# Autodesk Inventor assembly: Top_Separator Assy 3 Lanes
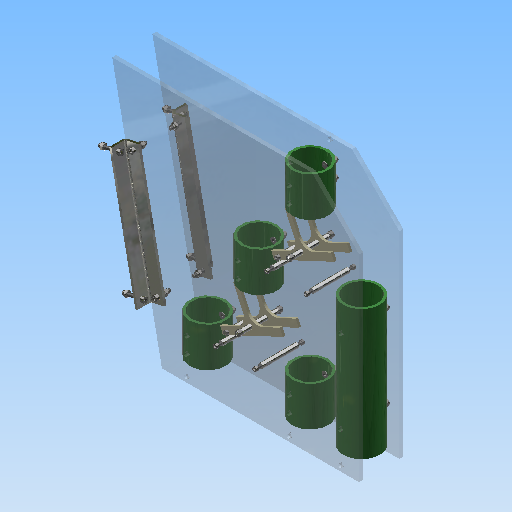
[picture p0: Inventor's stored thumbnail of the model, 512x512]
Saved by Autodesk Inventor 2018.1 (Build 221171000, 171)
## iProperties
Created: 2019-03-20
Part Number: Top_Separator Assy 3 Lanes
Document SubType Name: Assembly
Designer: James
Author: James
## Documents named in this file (16)
- C:\Users\admin\Desktop\Ball-Machine\Top Level\Top_Separator Assy 3 Lanes.iam
- C:\Users\admin\Desktop\Ball-Machine\Top Level\Top_Separator Pipe.ipt
- C:\Users\admin\Desktop\Ball-Machine\Top Level\Nyloc Nut - M4.ipt
- C:\Users\admin\Desktop\Ball-Machine\Top Level\Socket Csk Screw - (A2) - M4 x  16.ipt
- C:\Users\admin\Desktop\Ball-Machine\Pancake Sort\Pancake_Bearing.ipt
- C:\Users\admin\Desktop\Ball-Machine\Top Level\Top_Separator Shaft.ipt
- C:\Users\admin\Desktop\Ball-Machine\Timing Gate\BS 3673 - 6mm External Circlip.ipt
- C:\Users\admin\Desktop\Ball-Machine\Top Level\Top_Separator Lever.ipt
- C:\Users\admin\Desktop\Ball-Machine\Top Level\Top_Separator Weight.ipt
- C:\Users\admin\Desktop\Ball-Machine\Top Level\Socket Cap Screw - Standard - (A2) - M3 x 8.ipt
- C:\Users\admin\Desktop\Ball-Machine\Top Level\Top_Separator Weight 2.ipt
- C:\Users\admin\Desktop\Ball-Machine\Top Level\Top_Angle Bracket.ipt
- C:\Users\admin\Desktop\Ball-Machine\Top Level\Socket Cap Screw - Standard - (A2) - M4 x 16.ipt
- C:\Users\admin\Desktop\Ball-Machine\Top Level\Socket Cap Screw - Standard - (A2) - M4 x 25.ipt
- C:\Users\admin\Desktop\Ball-Machine\Top Level\Top_Separator Backboard 3 Lanes.ipt
- C:\Users\admin\Desktop\Ball-Machine\Top Level\Top_Separator Pipe Long.ipt
## Components (77 placed, 15 different names)
1. Top_Separator Backboard 3 Lanes:1 — Flush:1, Flush:2, Flush:3, Mate:29, Mate:30, Mate:31, Mate:32, Tangent:1, Angle:1, Tangent:2, Mate:33, Mate:34, Mate:35, Mate:36, Tangent:3, Mate:37, Mate:38, Mate:39, Mate:40, Tangent:6, Tangent:7, Mate:45, Mate:46, Mate:47, Mate:48, Mate:49, Mate:50, Mate:51, Mate:62, Flush:22, Mate:98, Mate:99, Mate:100, Mate:102, Mate:105, Mate:106, Mate:145, Flush:32, Flush:34, Flush:35, Flush:36, Mate:201, Mate:202, Mate:203, Flush:42
2. Top_Separator Backboard 3 Lanes:2 — Flush:33, Flush:34, Flush:35, Flush:36, Tangent:14, Mate:198, Mate:199, Mate:200, Flush:41
3. Top_Separator Pipe:1 — Mate:3, Mate:4, Mate:29, Mate:30, Tangent:1, Angle:1, Tangent:14
4. Top_Separator Pipe:2 — Tangent:2, Mate:33, Mate:34
5. Top_Separator Pipe Long:1 — Tangent:3, Mate:37, Mate:38
6. Top_Separator Pipe:5 — Tangent:6, Mate:45, Mate:46
7. Top_Separator Pipe:6 — Tangent:7, Mate:47, Mate:48
8. Pancake_Bearing:1 — Mate:55, Mate:56, Mate:62, Flush:33
9. Pancake_Bearing:2 — Mate:54, Mate:57, Flush:22
10. Top_Separator Shaft:1 — Mate:54, Mate:55, Mate:56, Mate:57, Mate:58, Mate:59, Mate:60, Mate:61, Mate:63, Mate:64
11. BS 3673 - 6mm External Circlip:1 — Mate:58, Mate:61, Flush:21, Mate:66
12. BS 3673 - 6mm External Circlip:2 — Mate:59, Mate:60, Flush:21, Mate:65
13. Top_Separator Lever:1 — Mate:64, Flush:23, Mate:66, Mate:68, Mate:71
14. Top_Separator Lever:2 — Mate:63, Flush:23, Mate:65, Mate:67, Mate:69, Mate:70, Mate:73, Tangent:8, Tangent:9
15. Top_Separator Weight:1 — Mate:67, Mate:68, Mate:69, Mate:72
16. Top_Separator Weight 2:2 — Mate:74, Mate:75, Mate:76, Mate:77, Flush:24, Mate:98, Mate:99, Tangent:8
17. Top_Separator Weight 2:3 — Flush:24, Mate:100, Tangent:9
18. Top_Separator Weight 2:4 — Flush:25, Mate:102, Mate:106, Tangent:11
19. Top_Separator Weight 2:5 — Flush:25, Mate:105, Tangent:10
20. Pancake_Bearing:3
21. Pancake_Bearing:4 — Mate:145, Flush:32
22. Top_Separator Shaft:2
23. BS 3673 - 6mm External Circlip:3
24. BS 3673 - 6mm External Circlip:4
25. Top_Separator Lever:3 — Mate:205, Mate:206, Mate:208
26. Top_Separator Lever:4 — Tangent:10, Tangent:11, Mate:207
27. Top_Angle Bracket:1 — Mate:174, Mate:175, Mate:176, Mate:177, Mate:178, Mate:179, Mate:180, Mate:181, Mate:201, Flush:42
28. Nyloc Nut - M4:15 — Mate:166, Mate:169
29. Socket Cap Screw - Standard - (A2) - M4 x 16:1 — Mate:167, Mate:168, Mate:176, Mate:177, Mate:203
30. Socket Cap Screw - Standard - (A2) - M4 x 25:1 — Mate:166, Mate:169, Mate:174, Mate:175
31. Nyloc Nut - M4:16 — Mate:167, Mate:168
32. Nyloc Nut - M4:17
33. Socket Cap Screw - Standard - (A2) - M4 x 16:2 — Mate:179, Mate:180, Mate:202
34. Socket Cap Screw - Standard - (A2) - M4 x 25:2 — Mate:178, Mate:181
35. Nyloc Nut - M4:18
36. Top_Angle Bracket:2 — Mate:198, Flush:41
37. Nyloc Nut - M4:19
38. Socket Cap Screw - Standard - (A2) - M4 x 16:3 — Mate:199
39. Socket Cap Screw - Standard - (A2) - M4 x 25:3
40. Nyloc Nut - M4:20
41. Nyloc Nut - M4:21
42. Socket Cap Screw - Standard - (A2) - M4 x 16:4 — Mate:200
43. Socket Cap Screw - Standard - (A2) - M4 x 25:4
44. Nyloc Nut - M4:22
45. Top_Separator Weight:2 — Mate:205, Mate:206, Mate:209, Mate:210
46. Socket Cap Screw - Standard - (A2) - M3 x 8:15 — Mate:208, Mate:209
47. Socket Cap Screw - Standard - (A2) - M3 x 8:16 — Mate:207, Mate:210
48. Socket Cap Screw - Standard - (A2) - M3 x 8:10
49. Socket Cap Screw - Standard - (A2) - M3 x 8:9
50. Socket Cap Screw - Standard - (A2) - M3 x 8:8
51. Socket Cap Screw - Standard - (A2) - M3 x 8:7
52. Socket Cap Screw - Standard - (A2) - M3 x 8:6
53. Socket Cap Screw - Standard - (A2) - M3 x 8:5
54. Socket Cap Screw - Standard - (A2) - M3 x 8:4 — Mate:75, Mate:76
55. Socket Cap Screw - Standard - (A2) - M3 x 8:3 — Mate:74, Mate:77
56. Socket Cap Screw - Standard - (A2) - M3 x 8:2 — Mate:71, Mate:72
57. Socket Cap Screw - Standard - (A2) - M3 x 8:1 — Mate:70, Mate:73
58. Nyloc Nut - M4:1 — Mate:1, Flush:4, Mate:32
59. Socket Csk Screw - (A2) - M4 x  16:1 — Mate:1, Flush:4, Mate:4
60. Nyloc Nut - M4:2 — Mate:2, Flush:5, Mate:31
61. Socket Csk Screw - (A2) - M4 x  16:2 — Mate:2, Flush:5, Mate:3
62. Nyloc Nut - M4:3 — Mate:35
63. Socket Csk Screw - (A2) - M4 x  16:3
64. Nyloc Nut - M4:4 — Mate:36
65. Socket Csk Screw - (A2) - M4 x  16:4
66. Nyloc Nut - M4:5 — Mate:39
67. Socket Csk Screw - (A2) - M4 x  16:5
68. Nyloc Nut - M4:6 — Mate:40
69. Socket Csk Screw - (A2) - M4 x  16:6
70. Nyloc Nut - M4:9 — Flush:18, Mate:51
71. Socket Csk Screw - (A2) - M4 x  16:9
72. Nyloc Nut - M4:10 — Flush:18
73. Socket Csk Screw - (A2) - M4 x  16:10
74. Nyloc Nut - M4:11 — Mate:49
75. Socket Csk Screw - (A2) - M4 x  16:11
76. Nyloc Nut - M4:12 — Mate:50
77. Socket Csk Screw - (A2) - M4 x  16:12
## Relationships (178: Mate 139, Flush 28, Tangent 10, Angle 1)
- Flush:1: Top_Separator Backboard 3 Lanes:1
- Flush:2: Top_Separator Backboard 3 Lanes:1
- Flush:3: Top_Separator Backboard 3 Lanes:1
- Mate:1: Nyloc Nut - M4:1 ↔ Socket Csk Screw - (A2) - M4 x  16:1
- Flush:4 (10 mm): Nyloc Nut - M4:1 ↔ Socket Csk Screw - (A2) - M4 x  16:1
- Mate:2: Nyloc Nut - M4:2 ↔ Socket Csk Screw - (A2) - M4 x  16:2
- Flush:5 (10 mm): Nyloc Nut - M4:2 ↔ Socket Csk Screw - (A2) - M4 x  16:2
- Mate:3: Top_Separator Pipe:1 ↔ Socket Csk Screw - (A2) - M4 x  16:2
- Mate:4: Top_Separator Pipe:1 ↔ Socket Csk Screw - (A2) - M4 x  16:1
- [Mate]: Nyloc Nut - M4:3 ↔ Socket Csk Screw - (A2) - M4 x  16:3
- [Flush] (10 mm): Nyloc Nut - M4:3 ↔ Socket Csk Screw - (A2) - M4 x  16:3
- [Mate]: Nyloc Nut - M4:4 ↔ Socket Csk Screw - (A2) - M4 x  16:4
- [Flush] (10 mm): Nyloc Nut - M4:4 ↔ Socket Csk Screw - (A2) - M4 x  16:4
- [Mate]: Top_Separator Pipe:2 ↔ Socket Csk Screw - (A2) - M4 x  16:4
- [Mate]: Top_Separator Pipe:2 ↔ Socket Csk Screw - (A2) - M4 x  16:3
- [Mate]: Nyloc Nut - M4:5 ↔ Socket Csk Screw - (A2) - M4 x  16:5
- [Flush] (10 mm): Nyloc Nut - M4:5 ↔ Socket Csk Screw - (A2) - M4 x  16:5
- [Mate]: Nyloc Nut - M4:6 ↔ Socket Csk Screw - (A2) - M4 x  16:6
- [Flush] (10 mm): Nyloc Nut - M4:6 ↔ Socket Csk Screw - (A2) - M4 x  16:6
- [Mate]: Top_Separator Pipe Long:1 ↔ Socket Csk Screw - (A2) - M4 x  16:6
- [Mate]: Top_Separator Pipe Long:1 ↔ Socket Csk Screw - (A2) - M4 x  16:5
- [Mate]: Nyloc Nut - M4:9 ↔ Socket Csk Screw - (A2) - M4 x  16:9
- [Flush] (10 mm): Nyloc Nut - M4:9 ↔ Socket Csk Screw - (A2) - M4 x  16:9
- [Mate]: Nyloc Nut - M4:10 ↔ Socket Csk Screw - (A2) - M4 x  16:10
- [Flush] (10 mm): Nyloc Nut - M4:10 ↔ Socket Csk Screw - (A2) - M4 x  16:10
- [Mate]: Top_Separator Pipe:5 ↔ Socket Csk Screw - (A2) - M4 x  16:10
- [Mate]: Top_Separator Pipe:5 ↔ Socket Csk Screw - (A2) - M4 x  16:9
- [Mate]: Nyloc Nut - M4:11 ↔ Socket Csk Screw - (A2) - M4 x  16:11
- [Flush] (10 mm): Nyloc Nut - M4:11 ↔ Socket Csk Screw - (A2) - M4 x  16:11
- [Mate]: Nyloc Nut - M4:12 ↔ Socket Csk Screw - (A2) - M4 x  16:12
- [Flush] (10 mm): Nyloc Nut - M4:12 ↔ Socket Csk Screw - (A2) - M4 x  16:12
- [Mate]: Top_Separator Pipe:6 ↔ Socket Csk Screw - (A2) - M4 x  16:12
- [Mate]: Top_Separator Pipe:6 ↔ Socket Csk Screw - (A2) - M4 x  16:11
- Mate:29: Top_Separator Backboard 3 Lanes:1 ↔ Top_Separator Pipe:1
- Mate:30: Top_Separator Backboard 3 Lanes:1 ↔ Top_Separator Pipe:1
- Mate:31: Top_Separator Backboard 3 Lanes:1 ↔ Nyloc Nut - M4:2
- Mate:32: Top_Separator Backboard 3 Lanes:1 ↔ Nyloc Nut - M4:1
- Tangent:1: Top_Separator Backboard 3 Lanes:1 ↔ Top_Separator Pipe:1
- Angle:1 (0 deg): Top_Separator Backboard 3 Lanes:1 ↔ Top_Separator Pipe:1
- Tangent:2: Top_Separator Backboard 3 Lanes:1 ↔ Top_Separator Pipe:2
- Mate:33: Top_Separator Backboard 3 Lanes:1 ↔ Top_Separator Pipe:2
- Mate:34: Top_Separator Backboard 3 Lanes:1 ↔ Top_Separator Pipe:2
- Mate:35: Top_Separator Backboard 3 Lanes:1 ↔ Nyloc Nut - M4:3
- Mate:36: Top_Separator Backboard 3 Lanes:1 ↔ Nyloc Nut - M4:4
- Tangent:3: Top_Separator Backboard 3 Lanes:1 ↔ Top_Separator Pipe Long:1
- Mate:37: Top_Separator Backboard 3 Lanes:1 ↔ Top_Separator Pipe Long:1
- Mate:38: Top_Separator Backboard 3 Lanes:1 ↔ Top_Separator Pipe Long:1
- Mate:39: Top_Separator Backboard 3 Lanes:1 ↔ Nyloc Nut - M4:5
- Mate:40: Top_Separator Backboard 3 Lanes:1 ↔ Nyloc Nut - M4:6
- Tangent:6: Top_Separator Backboard 3 Lanes:1 ↔ Top_Separator Pipe:5
- Tangent:7: Top_Separator Backboard 3 Lanes:1 ↔ Top_Separator Pipe:6
- Mate:45: Top_Separator Backboard 3 Lanes:1 ↔ Top_Separator Pipe:5
- Mate:46: Top_Separator Backboard 3 Lanes:1 ↔ Top_Separator Pipe:5
- Mate:47: Top_Separator Backboard 3 Lanes:1 ↔ Top_Separator Pipe:6
- Mate:48: Top_Separator Backboard 3 Lanes:1 ↔ Top_Separator Pipe:6
- Mate:49: Top_Separator Backboard 3 Lanes:1 ↔ Nyloc Nut - M4:11
- Mate:50: Top_Separator Backboard 3 Lanes:1 ↔ Nyloc Nut - M4:12
- Flush:18: Nyloc Nut - M4:9 ↔ Nyloc Nut - M4:10
- Mate:51: Top_Separator Backboard 3 Lanes:1 ↔ Nyloc Nut - M4:9
- Mate:54: Pancake_Bearing:2 ↔ Top_Separator Shaft:1
- Mate:55: Pancake_Bearing:1 ↔ Top_Separator Shaft:1
- Mate:56 (0.5 mm): Pancake_Bearing:1 ↔ Top_Separator Shaft:1
- Mate:57 (0.5 mm): Pancake_Bearing:2 ↔ Top_Separator Shaft:1
- Mate:58: Top_Separator Shaft:1 ↔ BS 3673 - 6mm External Circlip:1
- Mate:59: Top_Separator Shaft:1 ↔ BS 3673 - 6mm External Circlip:2
- Mate:60: Top_Separator Shaft:1 ↔ BS 3673 - 6mm External Circlip:2
- Mate:61: Top_Separator Shaft:1 ↔ BS 3673 - 6mm External Circlip:1
- Flush:21: BS 3673 - 6mm External Circlip:1 ↔ BS 3673 - 6mm External Circlip:2
- Mate:62: Top_Separator Backboard 3 Lanes:1 ↔ Pancake_Bearing:1
- Flush:22: Top_Separator Backboard 3 Lanes:1 ↔ Pancake_Bearing:2
- Mate:63: Top_Separator Shaft:1 ↔ Top_Separator Lever:2
- Mate:64: Top_Separator Shaft:1 ↔ Top_Separator Lever:1
- Flush:23: Top_Separator Lever:1 ↔ Top_Separator Lever:2
- Mate:65: BS 3673 - 6mm External Circlip:2 ↔ Top_Separator Lever:2
- Mate:66: BS 3673 - 6mm External Circlip:1 ↔ Top_Separator Lever:1
- Mate:67: Top_Separator Lever:2 ↔ Top_Separator Weight:1
- Mate:68: Top_Separator Lever:1 ↔ Top_Separator Weight:1
- Mate:69: Top_Separator Lever:2 ↔ Top_Separator Weight:1
- Mate:70: Top_Separator Lever:2 ↔ Socket Cap Screw - Standard - (A2) - M3 x 8:1
- Mate:71: Top_Separator Lever:1 ↔ Socket Cap Screw - Standard - (A2) - M3 x 8:2
- Mate:72: Top_Separator Weight:1 ↔ Socket Cap Screw - Standard - (A2) - M3 x 8:2
- Mate:73: Top_Separator Lever:2 ↔ Socket Cap Screw - Standard - (A2) - M3 x 8:1
- Mate:74: Top_Separator Weight 2:2 ↔ Socket Cap Screw - Standard - (A2) - M3 x 8:3
- Mate:75: Top_Separator Weight 2:2 ↔ Socket Cap Screw - Standard - (A2) - M3 x 8:4
- Mate:76 (5 mm): Top_Separator Weight 2:2 ↔ Socket Cap Screw - Standard - (A2) - M3 x 8:4
- Mate:77 (5 mm): Top_Separator Weight 2:2 ↔ Socket Cap Screw - Standard - (A2) - M3 x 8:3
- [Mate]: Top_Separator Weight 2:3 ↔ Socket Cap Screw - Standard - (A2) - M3 x 8:5
- [Mate]: Top_Separator Weight 2:3 ↔ Socket Cap Screw - Standard - (A2) - M3 x 8:6
- [Mate] (5 mm): Top_Separator Weight 2:3 ↔ Socket Cap Screw - Standard - (A2) - M3 x 8:6
- [Mate] (5 mm): Top_Separator Weight 2:3 ↔ Socket Cap Screw - Standard - (A2) - M3 x 8:5
- [Mate]: Top_Separator Weight 2:4 ↔ Socket Cap Screw - Standard - (A2) - M3 x 8:7
- [Mate]: Top_Separator Weight 2:4 ↔ Socket Cap Screw - Standard - (A2) - M3 x 8:8
- [Mate] (5 mm): Top_Separator Weight 2:4 ↔ Socket Cap Screw - Standard - (A2) - M3 x 8:8
- [Mate] (5 mm): Top_Separator Weight 2:4 ↔ Socket Cap Screw - Standard - (A2) - M3 x 8:7
- [Mate]: Top_Separator Weight 2:5 ↔ Socket Cap Screw - Standard - (A2) - M3 x 8:9
- [Mate]: Top_Separator Weight 2:5 ↔ Socket Cap Screw - Standard - (A2) - M3 x 8:10
- [Mate] (5 mm): Top_Separator Weight 2:5 ↔ Socket Cap Screw - Standard - (A2) - M3 x 8:10
- [Mate] (5 mm): Top_Separator Weight 2:5 ↔ Socket Cap Screw - Standard - (A2) - M3 x 8:9
- Flush:24: Top_Separator Weight 2:2 ↔ Top_Separator Weight 2:3
- Mate:98: Top_Separator Backboard 3 Lanes:1 ↔ Top_Separator Weight 2:2
- Mate:99: Top_Separator Backboard 3 Lanes:1 ↔ Top_Separator Weight 2:2
- Mate:100: Top_Separator Backboard 3 Lanes:1 ↔ Top_Separator Weight 2:3
- Flush:25: Top_Separator Weight 2:4 ↔ Top_Separator Weight 2:5
- Mate:102: Top_Separator Backboard 3 Lanes:1 ↔ Top_Separator Weight 2:4
- Mate:105: Top_Separator Backboard 3 Lanes:1 ↔ Top_Separator Weight 2:5
- Mate:106: Top_Separator Backboard 3 Lanes:1 ↔ Top_Separator Weight 2:4
- Tangent:8: Top_Separator Lever:2 ↔ Top_Separator Weight 2:2
- Tangent:9: Top_Separator Lever:2 ↔ Top_Separator Weight 2:3
- [Mate]: Pancake_Bearing:4 ↔ Top_Separator Shaft:2
- [Mate]: Pancake_Bearing:3 ↔ Top_Separator Shaft:2
- [Mate] (0.5 mm): Pancake_Bearing:3 ↔ Top_Separator Shaft:2
- [Mate] (0.5 mm): Pancake_Bearing:4 ↔ Top_Separator Shaft:2
- [Mate]: Top_Separator Shaft:2 ↔ BS 3673 - 6mm External Circlip:3
- [Mate]: Top_Separator Shaft:2 ↔ BS 3673 - 6mm External Circlip:4
- [Mate]: Top_Separator Shaft:2 ↔ BS 3673 - 6mm External Circlip:4
- [Mate]: Top_Separator Shaft:2 ↔ BS 3673 - 6mm External Circlip:3
- [Flush]: BS 3673 - 6mm External Circlip:3 ↔ BS 3673 - 6mm External Circlip:4
- [Mate]: Top_Separator Shaft:2 ↔ Top_Separator Lever:4
- [Mate]: Top_Separator Shaft:2 ↔ Top_Separator Lever:3
- [Flush]: Top_Separator Lever:3 ↔ Top_Separator Lever:4
- [Mate]: BS 3673 - 6mm External Circlip:4 ↔ Top_Separator Lever:4
- [Mate]: BS 3673 - 6mm External Circlip:3 ↔ Top_Separator Lever:3
- Mate:145: Top_Separator Backboard 3 Lanes:1 ↔ Pancake_Bearing:4
- Flush:32: Top_Separator Backboard 3 Lanes:1 ↔ Pancake_Bearing:4
- Tangent:10: Top_Separator Weight 2:5 ↔ Top_Separator Lever:4
- Tangent:11: Top_Separator Weight 2:4 ↔ Top_Separator Lever:4
- Flush:33: Top_Separator Backboard 3 Lanes:2 ↔ Pancake_Bearing:1
- Flush:34: Top_Separator Backboard 3 Lanes:1 ↔ Top_Separator Backboard 3 Lanes:2
- Flush:35: Top_Separator Backboard 3 Lanes:1 ↔ Top_Separator Backboard 3 Lanes:2
- Flush:36: Top_Separator Backboard 3 Lanes:1 ↔ Top_Separator Backboard 3 Lanes:2
- Tangent:14: Top_Separator Backboard 3 Lanes:2 ↔ Top_Separator Pipe:1
- Mate:166: Nyloc Nut - M4:15 ↔ Socket Cap Screw - Standard - (A2) - M4 x 25:1
- Mate:167: Socket Cap Screw - Standard - (A2) - M4 x 16:1 ↔ Nyloc Nut - M4:16
- Mate:168 (8 mm): Socket Cap Screw - Standard - (A2) - M4 x 16:1 ↔ Nyloc Nut - M4:16
- Mate:169 (18 mm): Nyloc Nut - M4:15 ↔ Socket Cap Screw - Standard - (A2) - M4 x 25:1
- [Mate]: Nyloc Nut - M4:17 ↔ Socket Cap Screw - Standard - (A2) - M4 x 25:2
- [Mate]: Socket Cap Screw - Standard - (A2) - M4 x 16:2 ↔ Nyloc Nut - M4:18
- [Mate] (8 mm): Socket Cap Screw - Standard - (A2) - M4 x 16:2 ↔ Nyloc Nut - M4:18
- [Mate] (18 mm): Nyloc Nut - M4:17 ↔ Socket Cap Screw - Standard - (A2) - M4 x 25:2
- Mate:174: Top_Angle Bracket:1 ↔ Socket Cap Screw - Standard - (A2) - M4 x 25:1
- Mate:175: Top_Angle Bracket:1 ↔ Socket Cap Screw - Standard - (A2) - M4 x 25:1
- Mate:176: Top_Angle Bracket:1 ↔ Socket Cap Screw - Standard - (A2) - M4 x 16:1
- Mate:177: Top_Angle Bracket:1 ↔ Socket Cap Screw - Standard - (A2) - M4 x 16:1
- Mate:178: Top_Angle Bracket:1 ↔ Socket Cap Screw - Standard - (A2) - M4 x 25:2
- Mate:179: Top_Angle Bracket:1 ↔ Socket Cap Screw - Standard - (A2) - M4 x 16:2
- Mate:180: Top_Angle Bracket:1 ↔ Socket Cap Screw - Standard - (A2) - M4 x 16:2
- Mate:181: Top_Angle Bracket:1 ↔ Socket Cap Screw - Standard - (A2) - M4 x 25:2
- [Mate]: Nyloc Nut - M4:19 ↔ Socket Cap Screw - Standard - (A2) - M4 x 25:3
- [Mate]: Socket Cap Screw - Standard - (A2) - M4 x 16:3 ↔ Nyloc Nut - M4:20
- [Mate] (8 mm): Socket Cap Screw - Standard - (A2) - M4 x 16:3 ↔ Nyloc Nut - M4:20
- [Mate] (18 mm): Nyloc Nut - M4:19 ↔ Socket Cap Screw - Standard - (A2) - M4 x 25:3
- [Mate]: Nyloc Nut - M4:21 ↔ Socket Cap Screw - Standard - (A2) - M4 x 25:4
- [Mate]: Socket Cap Screw - Standard - (A2) - M4 x 16:4 ↔ Nyloc Nut - M4:22
- [Mate] (8 mm): Socket Cap Screw - Standard - (A2) - M4 x 16:4 ↔ Nyloc Nut - M4:22
- [Mate] (18 mm): Nyloc Nut - M4:21 ↔ Socket Cap Screw - Standard - (A2) - M4 x 25:4
- [Mate]: Top_Angle Bracket:2 ↔ Socket Cap Screw - Standard - (A2) - M4 x 25:3
- [Mate]: Top_Angle Bracket:2 ↔ Socket Cap Screw - Standard - (A2) - M4 x 25:3
- [Mate]: Top_Angle Bracket:2 ↔ Socket Cap Screw - Standard - (A2) - M4 x 16:3
- [Mate]: Top_Angle Bracket:2 ↔ Socket Cap Screw - Standard - (A2) - M4 x 16:3
- [Mate]: Top_Angle Bracket:2 ↔ Socket Cap Screw - Standard - (A2) - M4 x 25:4
- [Mate]: Top_Angle Bracket:2 ↔ Socket Cap Screw - Standard - (A2) - M4 x 16:4
- [Mate]: Top_Angle Bracket:2 ↔ Socket Cap Screw - Standard - (A2) - M4 x 16:4
- [Mate]: Top_Angle Bracket:2 ↔ Socket Cap Screw - Standard - (A2) - M4 x 25:4
- Mate:198: Top_Separator Backboard 3 Lanes:2 ↔ Top_Angle Bracket:2
- Mate:199: Top_Separator Backboard 3 Lanes:2 ↔ Socket Cap Screw - Standard - (A2) - M4 x 16:3
- Mate:200: Top_Separator Backboard 3 Lanes:2 ↔ Socket Cap Screw - Standard - (A2) - M4 x 16:4
- Flush:41: Top_Separator Backboard 3 Lanes:2 ↔ Top_Angle Bracket:2
- Mate:201: Top_Separator Backboard 3 Lanes:1 ↔ Top_Angle Bracket:1
- Mate:202: Top_Separator Backboard 3 Lanes:1 ↔ Socket Cap Screw - Standard - (A2) - M4 x 16:2
- Mate:203: Top_Separator Backboard 3 Lanes:1 ↔ Socket Cap Screw - Standard - (A2) - M4 x 16:1
- Flush:42: Top_Separator Backboard 3 Lanes:1 ↔ Top_Angle Bracket:1
- [Mate]: Top_Separator Weight:2 ↔ Socket Cap Screw - Standard - (A2) - M3 x 8:16
- Mate:205: Top_Separator Lever:3 ↔ Top_Separator Weight:2
- Mate:206: Top_Separator Lever:3 ↔ Top_Separator Weight:2
- Mate:207: Top_Separator Lever:4 ↔ Socket Cap Screw - Standard - (A2) - M3 x 8:16
- Mate:208: Top_Separator Lever:3 ↔ Socket Cap Screw - Standard - (A2) - M3 x 8:15
- Mate:209: Top_Separator Weight:2 ↔ Socket Cap Screw - Standard - (A2) - M3 x 8:15
- Mate:210: Top_Separator Weight:2 ↔ Socket Cap Screw - Standard - (A2) - M3 x 8:16
## Named parameters: d9_d3 = 0 mm, d10_d4 = 10 mm, d11_d5 = 0 mm, d12_d6 = 10 mm, d13_d7 = 0 mm, d14_d8 = 0 mm, d15_d3 = 0 mm, d16_d4 = 10 mm, d17_d5 = 0 mm, d18_d6 = 10 mm, d19_d7 = 0 mm, d20_d8 = 0 mm, d27_d3 = 0 mm, d28_d4 = 10 mm, d29_d5 = 0 mm, d30_d6 = 10 mm, d31_d7 = 0 mm, d32_d8 = 0 mm, d33_d3 = 0 mm, d34_d4 = 10 mm, d35_d5 = 0 mm, d36_d6 = 10 mm, d37_d7 = 0 mm, d38_d8 = 0 mm, d108_d104 = 0 mm, d109_d105 = 0 mm, d110_d106 = 5 mm, d111_d107 = 5 mm, d112_d104 = 0 mm, d113_d105 = 0 mm, d114_d106 = 5 mm, d115_d107 = 5 mm, d116_d104 = 0 mm, d117_d105 = 0 mm, d118_d106 = 5 mm, d119_d107 = 5 mm, d152_d81 = 0 mm, d153_d82 = 0 mm, d154_d83 = 0.5 mm, d155_d84 = 0.5 mm, d156_d85 = 0 mm, d157_d86 = 0 mm, d158_d87 = 0 mm, d159_d88 = 0 mm, d160_d89 = 0 mm, d161_d92 = 0 mm, d162_d93 = 0 mm, d163_d94 = 0 mm, d164_d95 = 0 mm, d165_d96 = 0 mm, d236_d232 = 0 mm, d237_d233 = 0 mm, d238_d234 = 8 mm, d239_d235 = 18 mm, d248_d246 = 0 mm, d249_d247 = 0 mm, d250_d232 = 0 mm, d251_d233 = 0 mm, d252_d234 = 8 mm, d253_d235 = 18 mm, d254_d236_d232 = 0 mm, d255_d237_d233 = 0 mm, d256_d238_d234 = 8 mm, d257_d239_d235 = 18 mm, d258_d240 = 0 mm, d259_d241 = 0 mm, d260_d242 = 0 mm, d261_d243 = 0 mm, d262_d244 = 0 mm, d263_d245 = 0 mm, d272_d102 = 0 mm
